# Autodesk Inventor assembly: arm
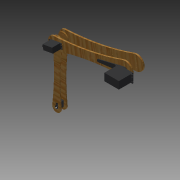
[picture p0: Inventor's stored thumbnail of the model, 180x180]
Saved by Autodesk Inventor 2013 (Build 170138000, 138)
## iProperties
Created: 2014-10-08
Part Number: arm
Document SubType Name: Assembly
Designer: Masta
Author: Masta
## Documents named in this file (4)
- D:\DrOctopus\3D model\arm.iam
- D:\DrOctopus\3D model\segment1.iam
- D:\DrOctopus\3D model\segment0.iam
- D:\DrOctopus\3D model\segment2.iam
## Components (3 placed, 3 different names)
1. segment1:1 [sub-assembly] — Insert:1, Insert:2
2. segment0:1 [sub-assembly] — Insert:1
3. segment2:1 [sub-assembly] — Insert:2
## Relationships (2: Insert 2)
- Insert:1: segment1:1 ↔ segment0:1
- Insert:2: segment1:1 ↔ segment2:1
